# Autodesk Inventor assembly: chess
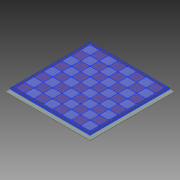
[picture p0: Inventor's stored thumbnail of the model, 180x180]
Saved by Autodesk Inventor 2013 SP1 (Build 170176100, 176)
## iProperties
Created: 2012-12-07
Part Number: chess
Document SubType Name: Assembly
Designer: Sebastian
Author: Sebastian
## Documents named in this file (4)
- E:\Projects\chess\construction\chess.iam
- E:\Projects\chess\construction\Spielfeld.ipt
- E:\Projects\chess\construction\_led.ipt
- E:\Projects\chess\construction\_platine.ipt
## Components (83 placed, 3 different names)
1. Spielfeld:1
2. platine:1
3. led:1
4. led:2
5. led:3
6. led:4
7. led:5
8. led:6
9. led:7
10. led:8
11. led:9
12. led:10
13. led:11
14. led:12
15. led:13
16. led:14
17. led:15
18. led:16
19. led:17
20. led:18
21. led:19
22. led:20
23. led:21
24. led:22
25. led:23
26. led:24
27. led:25
28. led:26
29. led:27
30. led:28
31. led:29
32. led:30
33. led:31
34. led:32
35. led:33
36. led:34
37. led:35
38. led:36
39. led:37
40. led:38
41. led:39
42. led:40
43. led:41
44. led:42
45. led:43
46. led:44
47. led:45
48. led:46
49. led:47
50. led:48
51. led:49
52. led:50
53. led:51
54. led:52
55. led:53
56. led:54
57. led:55
58. led:56
59. led:57
60. led:58
61. led:59
62. led:60
63. led:61
64. led:62
65. led:63
66. led:64
67. led:65
68. led:66
69. led:67
70. led:68
71. led:69
72. led:70
73. led:71
74. led:72
75. led:73
76. led:74
77. led:75
78. led:76
79. led:77
80. led:78
81. led:79
82. led:80
83. led:81
## Component patterns: (81 elements, first: led:1)
